# Autodesk Inventor assembly: Mold Design1
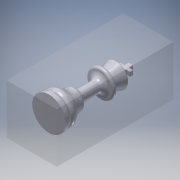
[picture p0: Inventor's stored thumbnail of the model, 180x180]
Saved by Autodesk Inventor 2018 (Build 220112000, 112)
## iProperties
Created: 2017-12-19
Part Number: Mold Design1
Document SubType Name: Assembly
Designer: 238438
Author: 238438
## Documents named in this file (2)
- P:\ied\chess\Mold Design1.iam
- P:\ied\chess\Mold Design1_Part1_LY.iam
## Components (1 placed, 1 different names)
1. Mold Design1_Part1_LY:1 [sub-assembly] — Flush:1, Flush:2, Flush:3
## Relationships (3: Flush 3)
- Flush:1: Mold Design1_Part1_LY:1
- Flush:2: Mold Design1_Part1_LY:1
- Flush:3: Mold Design1_Part1_LY:1
